# Autodesk Inventor assembly: SwerveDriveBracketASM
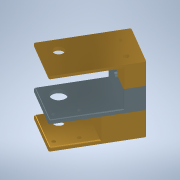
[picture p0: Inventor's stored thumbnail of the model, 180x180]
Saved by Autodesk Inventor 2022.3 (Build 263350000, 350)
## iProperties
Created: 2022-06-17
Part Number: SwerveDriveBracketASM
Document SubType Name: Assembly
Designer: Robert Nies
Author: Robert Nies
## Documents named in this file (4)
- C:\Users\rober\PycharmProjects\SwervoDrive\CAD\SwerveDriveBracketASM.iam
- C:\Users\rober\PycharmProjects\SwervoDrive\CAD\SwerveDriveBracket_A.ipt
- C:\Users\rober\PycharmProjects\SwervoDrive\CAD\SwerveDriveBracket_B.ipt
- C:\Users\rober\PycharmProjects\SwervoDrive\CAD\SwerveDriveBracket_C.ipt
## Components (3 placed, 3 different names)
1. SwerveDriveBracket_A:1 — Rotational:1, Rotational:2
2. SwerveDriveBracket_B:1 — Rotational:1, Rotational:2, Rotational:3, Rotational:4
3. SwerveDriveBracket_C:1 — Rotational:3, Rotational:4
## Relationships (4: RevoluteJoint 4)
- Rotational:1 [RevoluteJoint]: SwerveDriveBracket_A:1 ↔ SwerveDriveBracket_B:1
- Rotational:2 [RevoluteJoint]: SwerveDriveBracket_A:1 ↔ SwerveDriveBracket_B:1
- Rotational:3 [RevoluteJoint]: SwerveDriveBracket_B:1 ↔ SwerveDriveBracket_C:1
- Rotational:4 [RevoluteJoint]: SwerveDriveBracket_B:1 ↔ SwerveDriveBracket_C:1
